# Autodesk Inventor assembly: TowerAssembly
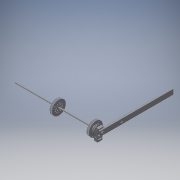
[picture p0: Inventor's stored thumbnail of the model, 180x180]
Saved by Autodesk Inventor 2018.3 (Build 223284000, 284)
## iProperties
Created: 2019-09-02
Part Number: TowerAssembly
Document SubType Name: Assembly
Designer: Srinity
Author: Srinity
## Documents named in this file (7)
- C:\Users\Srinity\Documents\DIY Projects\NerfGun\TowerAssembly.iam
- C:\Users\Srinity\Documents\DIY Projects\NerfGun\30inVersaFrameUpright.ipt
- C:\Users\Srinity\Documents\DIY Projects\NerfGun\13_75mm_1_2_ThunderHex_ID_x_1_125_OD_x_0_313_WD_Flanged_Bearing_217-4006 (1).ipt
- C:\Users\Srinity\Documents\DIY Projects\NerfGun\ThunderHex36.ipt
- C:\Users\Srinity\Documents\DIY Projects\NerfGun\Pulley with limit plates.iam
- C:\Users\Srinity\Documents\DIY Projects\NerfGun\45814-B.ipt
- C:\Users\Srinity\Documents\DIY Projects\NerfGun\RotateLimitSwitchHolder.ipt
## Components (7 placed, 6 different names)
1. 30inVersaFrameUpright:1 — Insert:1, Insert:2, Mate:2, Mate:3, Flush:1, Flush:3
2. 13_75mm_1_2_ThunderHex_ID_x_1_125_OD_x_0_313_WD_Flanged_Bearing_217-4006 (1):1 — Insert:2, Insert:3
3. 13_75mm_1_2_ThunderHex_ID_x_1_125_OD_x_0_313_WD_Flanged_Bearing_217-4006 (1):2 — Insert:1, Insert:4
4. ThunderHex36:1 — Insert:3, Mate:5, Mate:7
5. 45814-B:1 — Mate:5
6. RotateLimitSwitchHolder:1 — Insert:4, Flush:3, Mate:8
7. Pulley with limit plates:1 [sub-assembly] — Mate:7, Mate:8
## Relationships (11: Mate 5, Insert 4, Flush 2)
- Insert:1: 30inVersaFrameUpright:1 ↔ 13_75mm_1_2_ThunderHex_ID_x_1_125_OD_x_0_313_WD_Flanged_Bearing_217-4006 (1):2
- Insert:2: 30inVersaFrameUpright:1 ↔ 13_75mm_1_2_ThunderHex_ID_x_1_125_OD_x_0_313_WD_Flanged_Bearing_217-4006 (1):1
- Insert:3: 13_75mm_1_2_ThunderHex_ID_x_1_125_OD_x_0_313_WD_Flanged_Bearing_217-4006 (1):1 ↔ ThunderHex36:1
- Mate:2: 30inVersaFrameUpright:1
- Mate:3: 30inVersaFrameUpright:1
- Flush:1: 30inVersaFrameUpright:1
- Mate:5: ThunderHex36:1 ↔ 45814-B:1
- Insert:4: 13_75mm_1_2_ThunderHex_ID_x_1_125_OD_x_0_313_WD_Flanged_Bearing_217-4006 (1):2 ↔ RotateLimitSwitchHolder:1
- Flush:3: 30inVersaFrameUpright:1 ↔ RotateLimitSwitchHolder:1
- Mate:7: ThunderHex36:1 ↔ Pulley with limit plates:1
- Mate:8 (4.7625 mm): RotateLimitSwitchHolder:1 ↔ Pulley with limit plates:1
